# Autodesk Inventor assembly: futon completo
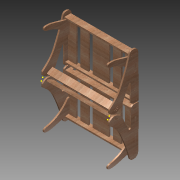
[picture p0: Inventor's stored thumbnail of the model, 180x180]
Saved by Autodesk Inventor 2015 (Build 190159000, 159)
## iProperties
Created: 2016-03-03
Part Number: futon completo
Document SubType Name: Assembly
Designer: iberopuebla
Author: iberopuebla
## Documents named in this file (2)
- C:\Users\iberopuebla.IBERO\Documents\Futón bien\futon completo.iam
- C:\Users\iberopuebla.IBERO\Documents\Futón bien\Assembly2.iam
## Components (2 placed, 1 different names)
1. Assembly2:1 [sub-assembly] — Mate:1, Mate:2, Mate:3, Mate:4, Mate:5
2. Assembly2:2 [sub-assembly] — Mate:1, Mate:2, Mate:3, Mate:4, Mate:5
## Relationships (5: Mate 5)
- Mate:1 (10 mm): Assembly2:1 ↔ Assembly2:2
- Mate:2 (10 mm): Assembly2:1 ↔ Assembly2:2
- Mate:3 (10 mm): Assembly2:1 ↔ Assembly2:2
- Mate:4 (10 mm): Assembly2:1 ↔ Assembly2:2
- Mate:5 (10 mm): Assembly2:1 ↔ Assembly2:2
